# Autodesk Inventor assembly: tenshoner ammebaly
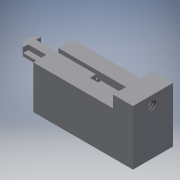
[picture p0: Inventor's stored thumbnail of the model, 180x180]
Saved by Autodesk Inventor 2019 (Build 230136000, 136)
## iProperties
Created: 2019-12-07
Part Number: tenshoner ammebaly
Document SubType Name: Assembly
Designer: User
Author: User
## Documents named in this file (3)
- C:\Robotics\CAD\2019-20_CAD\Collection\tenshoner ammebaly.iam
- C:\Robotics\CAD\2019-20_CAD\Collection\tenshoner base.ipt
- C:\Robotics\CAD\2019-20_CAD\Collection\tenshoner slider.ipt
## Components (2 placed, 2 different names)
1. tenshoner base:1 — Mate:1, Mate:2
2. tenshoner slider:1 — Mate:1, Mate:2
## Relationships (2: Mate 2)
- Mate:1 (0.3175 mm): tenshoner base:1 ↔ tenshoner slider:1
- Mate:2 (0.3175 mm): tenshoner base:1 ↔ tenshoner slider:1
